# Autodesk Inventor assembly: Assembly1
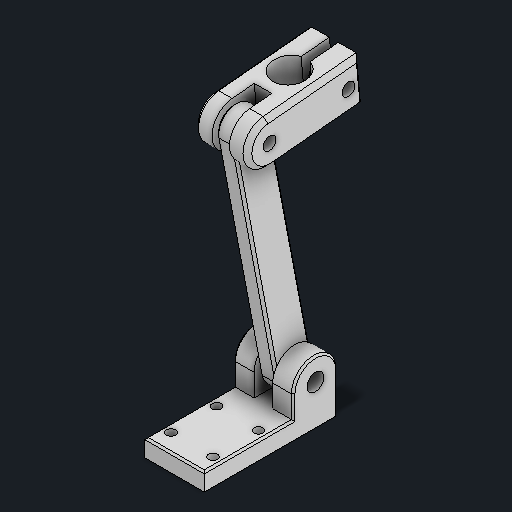
[picture p0: Inventor's stored thumbnail of the model, 512x512]
Saved by Autodesk Inventor 2025.1 (Build 291241020, 241B)
## iProperties
Created: 2025-05-04
Part Number: Assembly1
Document SubType Name: Assembly
Designer: Joshua Eah
Author: Joshua Eah
## Documents named in this file (4)
- C:\Users\Joshua Eah\Documents\GitHub\DesignedTrinkets\Dial Test Indicator\Assembly1.iam
- C:\Users\Joshua Eah\Documents\GitHub\DesignedTrinkets\Dial Test Indicator\Part1.ipt
- C:\Users\Joshua Eah\Documents\GitHub\DesignedTrinkets\Dial Test Indicator\Part2.ipt
- C:\Users\Joshua Eah\Documents\GitHub\DesignedTrinkets\Dial Test Indicator\Part3.ipt
## Components (3 placed, 3 different names)
1. Part1:1 — Rotational:2
2. Part2:1 — Rotational:1, Rotational:2
3. Part3:1 — Rotational:1
## Relationships (2: RevoluteJoint 2)
- Rotational:1 [RevoluteJoint]: Part2:1 ↔ Part3:1
- Rotational:2 [RevoluteJoint]: Part1:1 ↔ Part2:1
